# Autodesk Inventor assembly: Acquirer assembly v2
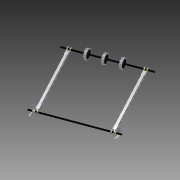
[picture p0: Inventor's stored thumbnail of the model, 180x180]
Saved by Autodesk Inventor 2014 SP1 (Build 180222100, 222)
## iProperties
Created: 2014-02-01
Part Number: Acquirer assembly v2
Document SubType Name: Assembly
Designer: Paul
Author: Paul
## Documents named in this file (8)
- C:\FRC_CAD\4859cad\Robot\Actual Robot\Acquire\Acquirer assembly v2.iam
- C:\FRC_CAD\4859cad\Robot\Actual Robot\Acquire\End Cap Bearing Mount.ipt
- C:\FRC_CAD\4859cad\Robot\Actual Robot\Acquire\Real Hex Bearing.ipt
- C:\FRC_CAD\4859cad\Robot\Actual Robot\Acquire\33 in hex shaft.ipt
- C:\FRC_CAD\4859cad\Robot\Actual Robot\Acquire\Corner Gusset.ipt
- C:\FRC_CAD\4859cad\Robot\Structure\Frame Assembly\1x1 tube 24in.ipt
- C:\FRC_CAD\4859cad\Robot\Actual Robot\Acquire\4 in wheel.iam
- C:\FRC_CAD\4859cad\Robot\Actual Robot\Acquire\500EX Hex wheel Hub.ipt
## Components (30 placed, 7 different names)
1. End Cap Bearing Mount:1 — Mate:33, Mate:34, Mate:80, Mate:81, Mate:82
2. End Cap Bearing Mount:2 — Mate:31, Mate:32, Flush:8, Mate:91, Mate:92, Mate:100
3. End Cap Bearing Mount:3 — Mate:37, Mate:38, Mate:86, Mate:87, Mate:99
4. End Cap Bearing Mount:4 — Mate:27, Mate:28, Mate:74, Mate:75, Mate:77
5. End Cap Bearing Mount:6 — Mate:25, Mate:26, Flush:8, Mate:76, Mate:79, Mate:117
6. End Cap Bearing Mount:7 — Mate:35, Mate:36, Mate:83, Mate:84, Mate:85
7. End Cap Bearing Mount:8 — Mate:39, Mate:40, Mate:88, Mate:89, Mate:90
8. Real Hex Bearing:1 — Mate:39, Mate:40, Flush:1, Flush:2
9. Real Hex Bearing:2 — Mate:37, Mate:38, Flush:1, Mate:102
10. Real Hex Bearing:3 — Mate:35, Mate:36, Flush:2, Flush:3
11. Real Hex Bearing:4 — Mate:33, Mate:34, Flush:3, Mate:43, Mate:44, Mate:104
12. Real Hex Bearing:6 — Mate:25, Mate:26, Rotation:1, Flush:6, Flush:7, Mate:42, Mate:120
13. Real Hex Bearing:7 — Mate:31, Mate:32, Flush:7
14. Real Hex Bearing:8 — Mate:27, Mate:28, Rotation:1, Flush:6, Mate:41, Mate:78
15. 33 in hex shaft:1 — Mate:41, Mate:42, Mate:78, Flush:14
16. 33 in hex shaft:2 — Mate:43, Mate:44, Flush:10, Mate:101, Mate:103, Flush:13
17. 1x1 tube 24in:1 — Mate:74, Mate:75, Mate:76, Mate:77, Mate:79, Mate:80, Mate:81, Mate:82, Mate:83, Mate:84, Mate:85, Flush:13, Flush:14
18. 1x1 tube 24in:2 — Mate:86, Mate:87, Mate:88, Mate:89, Mate:90, Mate:91, Mate:92, Mate:93, Mate:94, Mate:95, Mate:99, Mate:100, Flush:10
19. End Cap Bearing Mount:9 — Mate:93, Mate:94, Mate:95, Mate:96, Mate:97
20. Real Hex Bearing:11 — Mate:96, Mate:97
21. Corner Gusset:3 — Mate:101, Mate:102, Flush:12, Mate:105, Mate:106
22. Corner Gusset:4 — Mate:103, Mate:104, Flush:12, Mate:107, Mate:108
23. Real Hex Bearing:12 — Mate:105, Mate:106
24. Real Hex Bearing:13 — Mate:107, Mate:108
25. 4 in wheel:2 [sub-assembly] — Mate:112, Mate:115, Mate:119, Mate:122
26. 4 in wheel:3 [sub-assembly] — Mate:111, Mate:114, Mate:117, Mate:118, Mate:120, Mate:121
27. 4 in wheel:4 [sub-assembly] — Mate:113, Mate:116, Mate:118, Mate:119, Mate:121, Mate:122
28. 500EX Hex wheel Hub:2 — Mate:111, Mate:114
29. 500EX Hex wheel Hub:3 — Mate:112, Mate:115
30. 500EX Hex wheel Hub:4 — Mate:113, Mate:116
## Relationships (75: Mate 64, Flush 10, RelateRotation 1)
- Mate:25: End Cap Bearing Mount:6 ↔ Real Hex Bearing:6
- Mate:26: End Cap Bearing Mount:6 ↔ Real Hex Bearing:6
- Mate:27: End Cap Bearing Mount:4 ↔ Real Hex Bearing:8
- Mate:28: End Cap Bearing Mount:4 ↔ Real Hex Bearing:8
- Mate:31: End Cap Bearing Mount:2 ↔ Real Hex Bearing:7
- Mate:32: End Cap Bearing Mount:2 ↔ Real Hex Bearing:7
- Mate:33: End Cap Bearing Mount:1 ↔ Real Hex Bearing:4
- Mate:34: End Cap Bearing Mount:1 ↔ Real Hex Bearing:4
- Mate:35: End Cap Bearing Mount:7 ↔ Real Hex Bearing:3
- Mate:36: End Cap Bearing Mount:7 ↔ Real Hex Bearing:3
- Mate:37: End Cap Bearing Mount:3 ↔ Real Hex Bearing:2
- Mate:38: End Cap Bearing Mount:3 ↔ Real Hex Bearing:2
- Mate:39: End Cap Bearing Mount:8 ↔ Real Hex Bearing:1
- Mate:40: End Cap Bearing Mount:8 ↔ Real Hex Bearing:1
- Flush:1: Real Hex Bearing:1 ↔ Real Hex Bearing:2
- Flush:2: Real Hex Bearing:1 ↔ Real Hex Bearing:3
- Flush:3: Real Hex Bearing:3 ↔ Real Hex Bearing:4
- Rotation:1 [RelateRotation] (1 ul): Real Hex Bearing:6 ↔ Real Hex Bearing:8
- Flush:6: Real Hex Bearing:6 ↔ Real Hex Bearing:8
- Flush:7: Real Hex Bearing:6 ↔ Real Hex Bearing:7
- Mate:41: Real Hex Bearing:8 ↔ 33 in hex shaft:1
- Mate:42: Real Hex Bearing:6 ↔ 33 in hex shaft:1
- Flush:8: End Cap Bearing Mount:2 ↔ End Cap Bearing Mount:6
- Mate:43: Real Hex Bearing:4 ↔ 33 in hex shaft:2
- Mate:44: Real Hex Bearing:4 ↔ 33 in hex shaft:2
- Mate:74: End Cap Bearing Mount:4 ↔ 1x1 tube 24in:1
- Mate:75: End Cap Bearing Mount:4 ↔ 1x1 tube 24in:1
- Mate:76: End Cap Bearing Mount:6 ↔ 1x1 tube 24in:1
- Mate:77: End Cap Bearing Mount:4 ↔ 1x1 tube 24in:1
- Mate:78: Real Hex Bearing:8 ↔ 33 in hex shaft:1
- Mate:79: End Cap Bearing Mount:6 ↔ 1x1 tube 24in:1
- Mate:80: End Cap Bearing Mount:1 ↔ 1x1 tube 24in:1
- Mate:81: End Cap Bearing Mount:1 ↔ 1x1 tube 24in:1
- Mate:82: End Cap Bearing Mount:1 ↔ 1x1 tube 24in:1
- Mate:83: End Cap Bearing Mount:7 ↔ 1x1 tube 24in:1
- Mate:84: End Cap Bearing Mount:7 ↔ 1x1 tube 24in:1
- Mate:85: End Cap Bearing Mount:7 ↔ 1x1 tube 24in:1
- Mate:86: End Cap Bearing Mount:3 ↔ 1x1 tube 24in:2
- Mate:87: End Cap Bearing Mount:3 ↔ 1x1 tube 24in:2
- Mate:88: End Cap Bearing Mount:8 ↔ 1x1 tube 24in:2
- Mate:89: End Cap Bearing Mount:8 ↔ 1x1 tube 24in:2
- Mate:90: End Cap Bearing Mount:8 ↔ 1x1 tube 24in:2
- Mate:91: End Cap Bearing Mount:2 ↔ 1x1 tube 24in:2
- Mate:92: End Cap Bearing Mount:2 ↔ 1x1 tube 24in:2
- Mate:93: 1x1 tube 24in:2 ↔ End Cap Bearing Mount:9
- Mate:94: 1x1 tube 24in:2 ↔ End Cap Bearing Mount:9
- Mate:95: 1x1 tube 24in:2 ↔ End Cap Bearing Mount:9
- Mate:96: End Cap Bearing Mount:9 ↔ Real Hex Bearing:11
- Mate:97: End Cap Bearing Mount:9 ↔ Real Hex Bearing:11
- Mate:99: End Cap Bearing Mount:3 ↔ 1x1 tube 24in:2
- Mate:100: End Cap Bearing Mount:2 ↔ 1x1 tube 24in:2
- Flush:10 (63.5 mm): 33 in hex shaft:2 ↔ 1x1 tube 24in:2
- Mate:101 (-50.8 mm): 33 in hex shaft:2 ↔ Corner Gusset:3
- Mate:102: Real Hex Bearing:2 ↔ Corner Gusset:3
- Mate:103 (-50.8 mm): 33 in hex shaft:2 ↔ Corner Gusset:4
- Mate:104: Real Hex Bearing:4 ↔ Corner Gusset:4
- Flush:12: Corner Gusset:3 ↔ Corner Gusset:4
- Mate:105: Corner Gusset:3 ↔ Real Hex Bearing:12
- Mate:106: Corner Gusset:3 ↔ Real Hex Bearing:12
- Mate:107: Corner Gusset:4 ↔ Real Hex Bearing:13
- Mate:108: Corner Gusset:4 ↔ Real Hex Bearing:13
- Mate:111: 4 in wheel:3 ↔ 500EX Hex wheel Hub:2
- Mate:112: 4 in wheel:2 ↔ 500EX Hex wheel Hub:3
- Mate:113: 4 in wheel:4 ↔ 500EX Hex wheel Hub:4
- Mate:114: 4 in wheel:3 ↔ 500EX Hex wheel Hub:2
- Mate:115: 4 in wheel:2 ↔ 500EX Hex wheel Hub:3
- Mate:116: 4 in wheel:4 ↔ 500EX Hex wheel Hub:4
- Flush:13 (63.5 mm): 33 in hex shaft:2 ↔ 1x1 tube 24in:1
- Flush:14 (63.5 mm): 33 in hex shaft:1 ↔ 1x1 tube 24in:1
- Mate:117 (133.35 mm): End Cap Bearing Mount:6 ↔ 4 in wheel:3
- Mate:118 (133.35 mm): 4 in wheel:3 ↔ 4 in wheel:4
- Mate:119 (133.35 mm): 4 in wheel:2 ↔ 4 in wheel:4
- Mate:120: Real Hex Bearing:6 ↔ 4 in wheel:3
- Mate:121: 4 in wheel:3 ↔ 4 in wheel:4
- Mate:122: 4 in wheel:2 ↔ 4 in wheel:4
